# Autodesk Inventor assembly: CL6-p-100
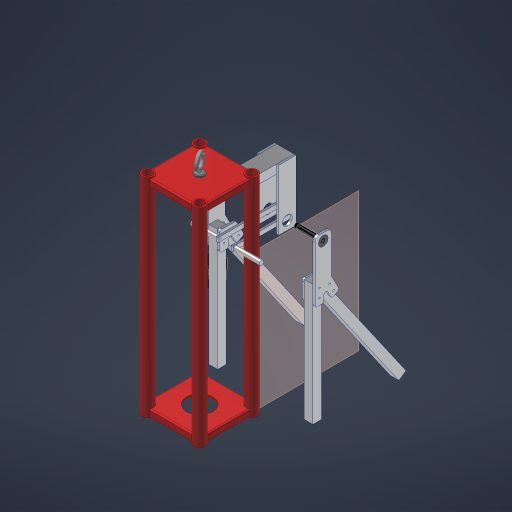
[picture p0: Inventor's stored thumbnail of the model, 512x512]
Saved by Autodesk Inventor 2023.4 (Build 274418000, 418)
## iProperties
Created: 2025-02-04
Part Number: CL6-p-100
Document SubType Name: Assembly
Designer: brand
Mass: 3247.43 g
Surface Area: 7567.76 cm^2
Volume: 1278.12 cm^3
Author: brand
## Documents named in this file (15)
- C:\Users\brand\OneDrive\Documents\GitHub\robotics 23\2025-ReefScape---CAD\Climber\CL6\CL6-p-100.iam
- C:\Users\brand\OneDrive\Documents\GitHub\robotics 23\2025-ReefScape---CAD\Climber\CL4\CL4-011.ipt
- C:\Users\brand\OneDrive\Documents\GitHub\robotics 23\2025-ReefScape---CAD\COMMON PARTS\BEARINGS\0_500_ID_x_1_125_OD_x_0_313_WD_Flanged_Bearing_217-2731.ipt
- C:\Users\brand\OneDrive\Documents\GitHub\robotics 23\2025-ReefScape---CAD\COMMON PARTS\ELECTRONICS\cameras\ELP Camera Angled' 17.5 + 7.5 deg up Case.ipt
- C:\Users\brand\OneDrive\Documents\GitHub\robotics 23\2025-ReefScape---CAD\Field Items\Full Field\FE-2025\GE-25201.iam
- C:\Users\brand\OneDrive\Documents\GitHub\robotics 23\2025-ReefScape---CAD\Climber\CL4\CL4-002.ipt
- C:\Users\brand\OneDrive\Documents\GitHub\robotics 23\2025-ReefScape---CAD\Climber\CL4\CL4-009.ipt
- C:\Users\brand\OneDrive\Documents\GitHub\robotics 23\2025-ReefScape---CAD\Climber\CL6\CL6-001.ipt
- C:\Users\brand\OneDrive\Documents\GitHub\robotics 23\2025-ReefScape---CAD\Climber\CL6\CL6-003.ipt
- C:\Users\brand\OneDrive\Documents\GitHub\robotics 23\2025-ReefScape---CAD\Climber\CL6\CL6-004.ipt
- C:\Users\brand\OneDrive\Documents\GitHub\robotics 23\2025-ReefScape---CAD\Climber\CL6\CL6-006.ipt
- C:\Users\brand\OneDrive\Documents\GitHub\robotics 23\2025-ReefScape---CAD\Climber\CL6\CL6-007.ipt
- C:\Users\brand\OneDrive\Documents\GitHub\robotics 23\2025-ReefScape---CAD\Field Items\Full Field\FE-2025\eyebolt_shoulder_.5_13_1.5.ipt
- C:\Users\brand\OneDrive\Documents\GitHub\robotics 23\2025-ReefScape---CAD\Field Items\Full Field\FE-2025\washer_flat_.5.ipt
- C:\Users\brand\OneDrive\Documents\GitHub\robotics 23\2025-ReefScape---CAD\Climber\CL6\CL6-P1.ipt
## Components (22 placed, 14 different names)
1. CL4-011:1 — Mate:19, Flush:2
2. 0_500_ID_x_1_125_OD_x_0_313_WD_Flanged_Bearing_217-2731:1
3. 0_500_ID_x_1_125_OD_x_0_313_WD_Flanged_Bearing_217-2731:2 — Mate:19, Flush:2, Mate:24
4. ELP Camera Angled' 17.5 + 7.5 deg up Case:2
5. GE-25201:1 [sub-assembly] — Insert:30, Mate:31, Flush:13, Mate:33
6. CL4-002:2 — Flush:14, Flush:15, Flush:16
7. CL4-009:1 — Insert:34, Flush:22
8. CL4-009:2 — Insert:32, Flush:20
9. CL6-001:1 — Insert:33, Flush:21, Angle:3
10. CL6-001:2 — Mate:28, Insert:31, Flush:19
11. CL6-003:1 — Mate:24, Mate:25, Angle:2, Mate:26, Flush:6, Flush:7, Mate:28, Mate:30
12. CL6-004:1 — Mate:26, Flush:6, Flush:7, Mate:27, Flush:12, Flush:13
13. CL6-003:2 — Mate:25, Angle:2, Mate:27, Mate:29, Flush:10, Flush:11, Mate:31, Angle:3
14. CL6-006:1 — Insert:26
15. CL6-006:2 — Insert:27
16. CL6-007:1 — Flush:8, Mate:29, Flush:9, Flush:10, Flush:11, Insert:26
17. CL6-007:2 — Flush:8, Mate:30, Flush:9, Insert:27
18. eyebolt_shoulder_.5_13_1.5:1 — Insert:29
19. washer_flat_.5:1 — Insert:28, Insert:29
20. washer_flat_.5:2 — Insert:28, Insert:30
21. CL6-P1:1 — Flush:17, Flush:18, Mate:32, Insert:33, Insert:34, Flush:21, Flush:22, Symmetry:1
22. CL6-P1:2 — Flush:14, Flush:15, Flush:16, Flush:17, Flush:18, Mate:32, Insert:31, Insert:32, Flush:19, Flush:20, Symmetry:1
## Relationships (47: Flush 18, Insert 14, Mate 12, Angle 2, Symmetry 1)
- [Insert]: 0_500_ID_x_1_125_OD_x_0_313_WD_Flanged_Bearing_217-2731:2 ↔ CL6-001:1
- [Insert]: 0_500_ID_x_1_125_OD_x_0_313_WD_Flanged_Bearing_217-2731:1 ↔ CL6-001:2
- Mate:19: CL4-011:1 ↔ 0_500_ID_x_1_125_OD_x_0_313_WD_Flanged_Bearing_217-2731:2
- Flush:2: CL4-011:1 ↔ 0_500_ID_x_1_125_OD_x_0_313_WD_Flanged_Bearing_217-2731:2
- [Insert]: ELP Camera Angled' 17.5 + 7.5 deg up Case:2 ↔ CL4-002:2
- [Insert]: ELP Camera Angled' 17.5 + 7.5 deg up Case:2 ↔ CL4-002:2
- [Insert]: CL4-002:2 ↔ CL6-001:2
- [Mate] (66.675 mm): CL6-001:1 ↔ CL6-001:2
- Mate:24: 0_500_ID_x_1_125_OD_x_0_313_WD_Flanged_Bearing_217-2731:2 ↔ CL6-003:1
- Mate:25: CL6-003:1 ↔ CL6-003:2
- Angle:2 (0 deg): CL6-003:1 ↔ CL6-003:2
- Mate:26: CL6-003:1 ↔ CL6-004:1
- Flush:6: CL6-003:1 ↔ CL6-004:1
- Flush:7: CL6-003:1 ↔ CL6-004:1
- Mate:27: CL6-004:1 ↔ CL6-003:2
- Mate:28: CL6-001:2 ↔ CL6-003:1
- Flush:8: CL6-007:1 ↔ CL6-007:2
- Mate:29: CL6-003:2 ↔ CL6-007:1
- Mate:30: CL6-003:1 ↔ CL6-007:2
- Flush:9: CL6-007:1 ↔ CL6-007:2
- Flush:10: CL6-003:2 ↔ CL6-007:1
- Flush:11 (19.05 mm): CL6-003:2 ↔ CL6-007:1
- Insert:26: CL6-006:1 ↔ CL6-007:1
- Insert:27: CL6-006:2 ↔ CL6-007:2
- Flush:12 (98.425 mm): CL6-004:1
- Insert:28: washer_flat_.5:1 ↔ washer_flat_.5:2
- Insert:29: eyebolt_shoulder_.5_13_1.5:1 ↔ washer_flat_.5:1
- Insert:30: GE-25201:1 ↔ washer_flat_.5:2
- Mate:31 (101.6 mm): GE-25201:1 ↔ CL6-003:2
- Flush:13 (-39.2176 mm): GE-25201:1 ↔ CL6-004:1
- Flush:14: CL4-002:2 ↔ CL6-P1:2
- Flush:15: CL4-002:2 ↔ CL6-P1:2
- Flush:16: CL4-002:2 ↔ CL6-P1:2
- Flush:17: CL6-P1:1 ↔ CL6-P1:2
- Flush:18: CL6-P1:1 ↔ CL6-P1:2
- Mate:32 (254 mm): CL6-P1:1 ↔ CL6-P1:2
- Insert:31: CL6-001:2 ↔ CL6-P1:2
- Insert:32: CL4-009:2 ↔ CL6-P1:2
- Flush:19: CL6-001:2 ↔ CL6-P1:2
- Flush:20: CL4-009:2 ↔ CL6-P1:2
- Insert:33: CL6-001:1 ↔ CL6-P1:1
- Insert:34: CL4-009:1 ↔ CL6-P1:1
- Flush:21: CL6-001:1 ↔ CL6-P1:1
- Flush:22: CL4-009:1 ↔ CL6-P1:1
- Symmetry:1: CL6-P1:1 ↔ CL6-P1:2
- Mate:33: GE-25201:1
- Angle:3 (0 deg): CL6-001:1 ↔ CL6-003:2
